# Autodesk Inventor assembly: Bumper Half Assembly
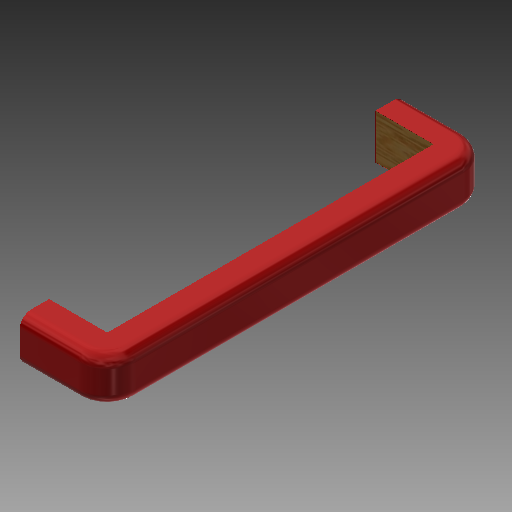
[picture p0: Inventor's stored thumbnail of the model, 512x512]
Saved by Autodesk Inventor 2019.4 (Build 234330000, 330)
## iProperties
Created: 2020-01-22
Part Number: Bumper Half Assembly
Document SubType Name: Assembly
Designer: admin
Surface Area: 17894.2 cm^2
Volume: 12477 cm^3
Author: admin
## Documents named in this file (4)
- C:\Users\Mark\Desktop\7738 Helion Engineering\7738-2020\Robot V2\Bumper\Bumper Half Assembly.iam
- C:\Users\Mark\Desktop\7738 Helion Engineering\7738-2020\Robot V2\Bumper\Bumper Wood 1.ipt
- C:\Users\Mark\Desktop\7738 Helion Engineering\7738-2020\Robot V2\Bumper\Bumper Wood 2.ipt
- C:\Users\Mark\Desktop\7738 Helion Engineering\7738-2020\Robot V2\Bumper\Bumper Fabric.ipt
## Components (4 placed, 3 different names)
1. Bumper Wood 1:1 — Mate:1, Flush:1, Flush:2, Mate:2, Flush:3, Flush:4
2. Bumper Wood 2:1 — Mate:1, Flush:1, Flush:2, Angle:1
3. Bumper Wood 2:2 — Mate:2, Flush:3, Flush:4
4. Bumper Fabric:1 — Angle:1
## Relationships (7: Flush 4, Mate 2, Angle 1)
- Mate:1: Bumper Wood 1:1 ↔ Bumper Wood 2:1
- Flush:1: Bumper Wood 1:1 ↔ Bumper Wood 2:1
- Flush:2: Bumper Wood 1:1 ↔ Bumper Wood 2:1
- Mate:2: Bumper Wood 1:1 ↔ Bumper Wood 2:2
- Flush:3: Bumper Wood 1:1 ↔ Bumper Wood 2:2
- Flush:4: Bumper Wood 1:1 ↔ Bumper Wood 2:2
- Angle:1 (0 deg): Bumper Wood 2:1 ↔ Bumper Fabric:1
